# Autodesk Inventor assembly: hipsAndLegs
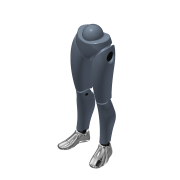
[picture p0: Inventor's stored thumbnail of the model, 180x180]
Saved by Autodesk Inventor 2018 (Build 220112000, 112)
## iProperties
Created: 2020-03-04
Part Number: hipsAndLegs
Document SubType Name: Assembly
Designer: Matt
Author: Matt
## Documents named in this file (2)
- C:\Users\Matt\robot\multibodySim\human\Corpo Humano - ADEBOTT Projetos\hipsAndLegs.iam
- C:\Users\Matt\robot\multibodySim\human\Corpo Humano - ADEBOTT Projetos\01.01.01.00 - Membros inferiores.iam
## Components (1 placed, 1 different names)
1. 01.01.01.00 - Membros inferiores:1 [sub-assembly] — Flush:1, Flush:2, Flush:3
## Relationships (3: Flush 3)
- Flush:1: 01.01.01.00 - Membros inferiores:1
- Flush:2 (1016 mm): 01.01.01.00 - Membros inferiores:1
- Flush:3 (6.35 mm): 01.01.01.00 - Membros inferiores:1
